# Autodesk Inventor assembly: SPE44V1 Acrilico Paciente
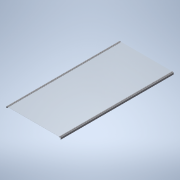
[picture p0: Inventor's stored thumbnail of the model, 180x180]
Saved by Autodesk Inventor 2021.2 (Build 252289000, 289)
## iProperties
Created: 2026-08-25
Part Number: SPE44V1 Acrilico Paciente
Document SubType Name: Assembly
Designer: nelso
Author: nelso
## Documents named in this file (8)
- C:\Users\nelso\Desktop\Soporte-Paciente-Espinografia\Workspace\SPE44V1 Acrilico Paciente.iam
- C:\Users\nelso\Desktop\Soporte-Paciente-Espinografia\Workspace\SP25V1 Acrilico.ipt
- C:\Users\nelso\Desktop\Soporte-Paciente-Espinografia\Workspace\SP28V1 Seguro Acrilico.ipt
- C:\Users\nelso\Desktop\Soporte-Paciente-Espinografia\Workspace\ISO7380M4X0.8L16I.ipt
- C:\Users\nelso\Desktop\Soporte-Paciente-Espinografia\Workspace\SP39V1 Chapa Acrilico.ipt
- C:\Users\nelso\Desktop\Soporte-Paciente-Espinografia\Workspace\DIN555-5M4X0.8I.ipt
- C:\Users\nelso\Desktop\Soporte-Paciente-Espinografia\Workspace\DIN125A4C.ipt
- C:\Users\nelso\Desktop\Soporte-Paciente-Espinografia\Workspace\SP47V1 Chapa Acrilico Pasador.ipt
## Components (56 placed, 7 different names)
1. SP25V1 Acrilico:1 — Mate:114, Mate:116
2. SP28V1 Seguro Acrilico:1
3. SP28V1 Seguro Acrilico:2
4. ISO7380M4X0.8L16I:1 — Mate:117
5. ISO7380M4X0.8L16I:2
6. ISO7380M4X0.8L16I:3
7. ISO7380M4X0.8L16I:4
8. ISO7380M4X0.8L16I:5
9. ISO7380M4X0.8L16I:7
10. ISO7380M4X0.8L16I:8
11. ISO7380M4X0.8L16I:9 — Mate:118
12. ISO7380M4X0.8L16I:10 — Mate:113, Mate:114
13. ISO7380M4X0.8L16I:11
14. ISO7380M4X0.8L16I:12
15. ISO7380M4X0.8L16I:13
16. ISO7380M4X0.8L16I:14
17. ISO7380M4X0.8L16I:15
18. ISO7380M4X0.8L16I:16
19. ISO7380M4X0.8L16I:17 — Mate:115
20. ISO7380M4X0.8L16I:18
21. SP39V1 Chapa Acrilico:1 — Mate:113, Mate:115
22. DIN555-5M4X0.8I:1
23. DIN555-5M4X0.8I:2
24. DIN555-5M4X0.8I:3
25. DIN555-5M4X0.8I:4
26. DIN555-5M4X0.8I:5
27. DIN555-5M4X0.8I:7
28. DIN555-5M4X0.8I:8
29. DIN555-5M4X0.8I:9
30. DIN555-5M4X0.8I:10
31. DIN555-5M4X0.8I:11
32. DIN555-5M4X0.8I:12
33. DIN555-5M4X0.8I:13
34. DIN555-5M4X0.8I:14
35. DIN555-5M4X0.8I:15
36. DIN555-5M4X0.8I:16
37. DIN555-5M4X0.8I:17
38. DIN555-5M4X0.8I:18
39. DIN125A4C:1
40. DIN125A4C:2
41. DIN125A4C:3
42. DIN125A4C:4
43. DIN125A4C:5
44. DIN125A4C:7
45. DIN125A4C:8
46. DIN125A4C:9
47. DIN125A4C:10
48. DIN125A4C:11
49. DIN125A4C:12
50. DIN125A4C:13
51. DIN125A4C:14
52. DIN125A4C:15
53. DIN125A4C:16
54. DIN125A4C:17
55. DIN125A4C:18
56. SP47V1 Chapa Acrilico Pasador:1 — Mate:116, Mate:117, Mate:118
## Relationships (106: Mate 103, Flush 3)
- [Mate]: SP25V1 Acrilico:1 ↔ SP28V1 Seguro Acrilico:1
- [Mate]: SP25V1 Acrilico:1 ↔ SP28V1 Seguro Acrilico:2
- [Flush]: SP25V1 Acrilico:1 ↔ SP28V1 Seguro Acrilico:1
- [Flush]: SP25V1 Acrilico:1 ↔ SP28V1 Seguro Acrilico:2
- [Mate]: SP28V1 Seguro Acrilico:1 ↔ ISO7380M4X0.8L16I:1
- [Mate]: SP28V1 Seguro Acrilico:1 ↔ ISO7380M4X0.8L16I:2
- [Mate]: SP28V1 Seguro Acrilico:1 ↔ ISO7380M4X0.8L16I:3
- [Mate]: SP28V1 Seguro Acrilico:1 ↔ ISO7380M4X0.8L16I:4
- [Mate]: SP28V1 Seguro Acrilico:1 ↔ ISO7380M4X0.8L16I:5
- [Mate]: SP28V1 Seguro Acrilico:1 ↔ ISO7380M4X0.8L16I:7
- [Mate]: SP28V1 Seguro Acrilico:1 ↔ ISO7380M4X0.8L16I:8
- [Mate]: SP28V1 Seguro Acrilico:1 ↔ ISO7380M4X0.8L16I:9
- [Mate]: SP28V1 Seguro Acrilico:2 ↔ ISO7380M4X0.8L16I:10
- [Mate]: SP28V1 Seguro Acrilico:2 ↔ ISO7380M4X0.8L16I:11
- [Mate]: SP28V1 Seguro Acrilico:2 ↔ ISO7380M4X0.8L16I:12
- [Mate]: SP28V1 Seguro Acrilico:2 ↔ ISO7380M4X0.8L16I:13
- [Mate]: SP28V1 Seguro Acrilico:2 ↔ ISO7380M4X0.8L16I:14
- [Mate]: SP28V1 Seguro Acrilico:2 ↔ ISO7380M4X0.8L16I:18
- [Mate]: SP28V1 Seguro Acrilico:2 ↔ ISO7380M4X0.8L16I:15
- [Mate]: SP28V1 Seguro Acrilico:2 ↔ ISO7380M4X0.8L16I:16
- [Mate]: SP28V1 Seguro Acrilico:2 ↔ ISO7380M4X0.8L16I:17
- [Mate]: SP28V1 Seguro Acrilico:1 ↔ ISO7380M4X0.8L16I:1
- [Mate]: SP28V1 Seguro Acrilico:1 ↔ ISO7380M4X0.8L16I:2
- [Mate]: SP28V1 Seguro Acrilico:1 ↔ ISO7380M4X0.8L16I:3
- [Mate]: SP28V1 Seguro Acrilico:1 ↔ ISO7380M4X0.8L16I:4
- [Mate]: SP28V1 Seguro Acrilico:1 ↔ ISO7380M4X0.8L16I:5
- [Mate]: SP28V1 Seguro Acrilico:1 ↔ ISO7380M4X0.8L16I:7
- [Mate]: SP28V1 Seguro Acrilico:1 ↔ ISO7380M4X0.8L16I:8
- [Mate]: SP28V1 Seguro Acrilico:1 ↔ ISO7380M4X0.8L16I:9
- [Mate]: SP28V1 Seguro Acrilico:2 ↔ ISO7380M4X0.8L16I:16
- [Mate]: SP28V1 Seguro Acrilico:2 ↔ ISO7380M4X0.8L16I:15
- [Mate]: SP28V1 Seguro Acrilico:2 ↔ ISO7380M4X0.8L16I:18
- [Mate]: SP28V1 Seguro Acrilico:2 ↔ ISO7380M4X0.8L16I:14
- [Mate]: SP28V1 Seguro Acrilico:2 ↔ ISO7380M4X0.8L16I:13
- [Mate]: SP28V1 Seguro Acrilico:2 ↔ ISO7380M4X0.8L16I:11
- [Mate]: SP25V1 Acrilico:1 ↔ SP39V1 Chapa Acrilico:1
- [Flush]: SP25V1 Acrilico:1 ↔ SP28V1 Seguro Acrilico:1
- [Mate]: ISO7380M4X0.8L16I:1 ↔ DIN555-5M4X0.8I:1
- [Mate]: ISO7380M4X0.8L16I:2 ↔ DIN555-5M4X0.8I:2
- [Mate]: ISO7380M4X0.8L16I:3 ↔ DIN555-5M4X0.8I:3
- [Mate]: ISO7380M4X0.8L16I:4 ↔ DIN555-5M4X0.8I:4
- [Mate]: ISO7380M4X0.8L16I:5 ↔ DIN555-5M4X0.8I:5
- [Mate]: ISO7380M4X0.8L16I:7 ↔ DIN555-5M4X0.8I:7
- [Mate]: ISO7380M4X0.8L16I:8 ↔ DIN555-5M4X0.8I:8
- [Mate]: ISO7380M4X0.8L16I:9 ↔ DIN555-5M4X0.8I:9
- [Mate]: ISO7380M4X0.8L16I:10 ↔ DIN555-5M4X0.8I:10
- [Mate]: ISO7380M4X0.8L16I:11 ↔ DIN555-5M4X0.8I:11
- [Mate]: ISO7380M4X0.8L16I:12 ↔ DIN555-5M4X0.8I:12
- [Mate]: ISO7380M4X0.8L16I:13 ↔ DIN555-5M4X0.8I:13
- [Mate]: ISO7380M4X0.8L16I:14 ↔ DIN555-5M4X0.8I:14
- [Mate]: ISO7380M4X0.8L16I:18 ↔ DIN555-5M4X0.8I:15
- [Mate]: ISO7380M4X0.8L16I:15 ↔ DIN555-5M4X0.8I:16
- [Mate]: ISO7380M4X0.8L16I:16 ↔ DIN555-5M4X0.8I:17
- [Mate]: ISO7380M4X0.8L16I:17 ↔ DIN555-5M4X0.8I:18
- [Mate]: ISO7380M4X0.8L16I:10 ↔ DIN125A4C:18
- [Mate]: ISO7380M4X0.8L16I:11 ↔ DIN125A4C:17
- [Mate]: ISO7380M4X0.8L16I:12 ↔ DIN125A4C:16
- [Mate]: ISO7380M4X0.8L16I:13 ↔ DIN125A4C:15
- [Mate]: ISO7380M4X0.8L16I:14 ↔ DIN125A4C:14
- [Mate]: ISO7380M4X0.8L16I:18 ↔ DIN125A4C:13
- [Mate]: ISO7380M4X0.8L16I:15 ↔ DIN125A4C:12
- [Mate]: ISO7380M4X0.8L16I:17 ↔ DIN125A4C:11
- [Mate]: ISO7380M4X0.8L16I:16 ↔ DIN125A4C:10
- [Mate]: ISO7380M4X0.8L16I:9 ↔ DIN125A4C:9
- [Mate]: ISO7380M4X0.8L16I:8 ↔ DIN125A4C:8
- [Mate]: ISO7380M4X0.8L16I:7 ↔ DIN125A4C:7
- [Mate]: ISO7380M4X0.8L16I:5 ↔ DIN125A4C:5
- [Mate]: ISO7380M4X0.8L16I:4 ↔ DIN125A4C:4
- [Mate]: ISO7380M4X0.8L16I:3 ↔ DIN125A4C:3
- [Mate]: ISO7380M4X0.8L16I:2 ↔ DIN125A4C:2
- [Mate]: ISO7380M4X0.8L16I:1 ↔ DIN125A4C:1
- [Mate]: DIN555-5M4X0.8I:1 ↔ DIN125A4C:1
- [Mate]: DIN555-5M4X0.8I:2 ↔ DIN125A4C:2
- [Mate]: DIN555-5M4X0.8I:3 ↔ DIN125A4C:3
- [Mate]: DIN555-5M4X0.8I:4 ↔ DIN125A4C:4
- [Mate]: DIN555-5M4X0.8I:5 ↔ DIN125A4C:5
- [Mate]: DIN555-5M4X0.8I:7 ↔ DIN125A4C:7
- [Mate]: DIN555-5M4X0.8I:8 ↔ DIN125A4C:8
- [Mate]: DIN555-5M4X0.8I:9 ↔ DIN125A4C:9
- [Mate]: SP39V1 Chapa Acrilico:1 ↔ DIN125A4C:11
- [Mate]: DIN555-5M4X0.8I:18 ↔ DIN125A4C:11
- [Mate]: SP39V1 Chapa Acrilico:1 ↔ DIN125A4C:10
- [Mate]: DIN555-5M4X0.8I:17 ↔ DIN125A4C:10
- [Mate]: SP39V1 Chapa Acrilico:1 ↔ DIN125A4C:12
- [Mate]: DIN555-5M4X0.8I:16 ↔ DIN125A4C:12
- [Mate]: SP39V1 Chapa Acrilico:1 ↔ DIN125A4C:13
- [Mate]: DIN555-5M4X0.8I:15 ↔ DIN125A4C:13
- [Mate]: SP39V1 Chapa Acrilico:1 ↔ DIN125A4C:14
- [Mate]: DIN555-5M4X0.8I:14 ↔ DIN125A4C:14
- [Mate]: SP39V1 Chapa Acrilico:1 ↔ DIN125A4C:15
- [Mate]: DIN555-5M4X0.8I:13 ↔ DIN125A4C:15
- [Mate]: SP39V1 Chapa Acrilico:1 ↔ DIN125A4C:16
- [Mate]: DIN555-5M4X0.8I:12 ↔ DIN125A4C:16
- [Mate]: SP39V1 Chapa Acrilico:1 ↔ DIN125A4C:17
- [Mate]: DIN555-5M4X0.8I:11 ↔ DIN125A4C:17
- [Mate]: SP39V1 Chapa Acrilico:1 ↔ DIN125A4C:18
- [Mate]: DIN555-5M4X0.8I:10 ↔ DIN125A4C:18
- [Mate]: SP28V1 Seguro Acrilico:2 ↔ ISO7380M4X0.8L16I:17
- [Mate]: SP28V1 Seguro Acrilico:2 ↔ ISO7380M4X0.8L16I:10
- [Mate]: SP28V1 Seguro Acrilico:2 ↔ ISO7380M4X0.8L16I:12
- Mate:113: ISO7380M4X0.8L16I:10 ↔ SP39V1 Chapa Acrilico:1
- Mate:114: SP25V1 Acrilico:1 ↔ ISO7380M4X0.8L16I:10
- Mate:115: ISO7380M4X0.8L16I:17 ↔ SP39V1 Chapa Acrilico:1
- Mate:116: SP25V1 Acrilico:1 ↔ SP47V1 Chapa Acrilico Pasador:1
- Mate:117: ISO7380M4X0.8L16I:1 ↔ SP47V1 Chapa Acrilico Pasador:1
- Mate:118: ISO7380M4X0.8L16I:9 ↔ SP47V1 Chapa Acrilico Pasador:1
